# Autodesk Inventor assembly: 知能ロボコンターンテーブル合体.ipt
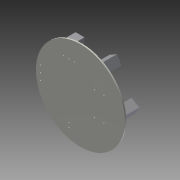
[picture p0: Inventor's stored thumbnail of the model, 180x180]
Saved by Autodesk Inventor 2013 (Build 170138000, 138)
## iProperties
Created: 2014-05-11
Part Number: 知能ロボコンターンテーブル合体.ipt
Document SubType Name: Assembly
Designer: horumo136
Author: horumo136
## Documents named in this file (3)
- C:\Users\horumo136\Documents\知能ロボコンターンテーブル合体.ipt.iam
- C:\Users\horumo136\Documents\知能ロボコンターンテーブル.ipt
- C:\Users\horumo136\Documents\知能ロボコンボールキャスタ.ipt
## Components (7 placed, 2 different names)
1. 知能ロボコンターンテーブル:1 — メイト:1, メイト:2, メイト:3, メイト:4, メイト:5, メイト:6, メイト:7, メイト:8, メイト:9, メイト:10, メイト:11, メイト:12, メイト:13, メイト:14
2. 知能ロボコンボールキャスタ:1 — メイト:7, メイト:8
3. 知能ロボコンボールキャスタ:2 — メイト:13, メイト:14
4. 知能ロボコンボールキャスタ:3 — メイト:9, メイト:10
5. 知能ロボコンボールキャスタ:4 — メイト:1, メイト:2, メイト:3
6. 知能ロボコンボールキャスタ:5 — メイト:11, メイト:12
7. 知能ロボコンボールキャスタ:6 — メイト:4, メイト:5, メイト:6
## Relationships (14: Mate 14)
- メイト:1 [Mate]: 知能ロボコンターンテーブル:1 ↔ 知能ロボコンボールキャスタ:4
- メイト:2 [Mate]: 知能ロボコンターンテーブル:1 ↔ 知能ロボコンボールキャスタ:4
- メイト:3 [Mate]: 知能ロボコンターンテーブル:1 ↔ 知能ロボコンボールキャスタ:4
- メイト:4 [Mate]: 知能ロボコンターンテーブル:1 ↔ 知能ロボコンボールキャスタ:6
- メイト:5 [Mate]: 知能ロボコンターンテーブル:1 ↔ 知能ロボコンボールキャスタ:6
- メイト:6 [Mate]: 知能ロボコンターンテーブル:1 ↔ 知能ロボコンボールキャスタ:6
- メイト:7 [Mate]: 知能ロボコンターンテーブル:1 ↔ 知能ロボコンボールキャスタ:1
- メイト:8 [Mate]: 知能ロボコンターンテーブル:1 ↔ 知能ロボコンボールキャスタ:1
- メイト:9 [Mate]: 知能ロボコンターンテーブル:1 ↔ 知能ロボコンボールキャスタ:3
- メイト:10 [Mate]: 知能ロボコンターンテーブル:1 ↔ 知能ロボコンボールキャスタ:3
- メイト:11 [Mate]: 知能ロボコンターンテーブル:1 ↔ 知能ロボコンボールキャスタ:5
- メイト:12 [Mate]: 知能ロボコンターンテーブル:1 ↔ 知能ロボコンボールキャスタ:5
- メイト:13 [Mate]: 知能ロボコンターンテーブル:1 ↔ 知能ロボコンボールキャスタ:2
- メイト:14 [Mate]: 知能ロボコンターンテーブル:1 ↔ 知能ロボコンボールキャスタ:2
